# Autodesk Inventor assembly: N_core
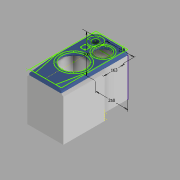
[picture p0: Inventor's stored thumbnail of the model, 180x180]
Saved by Autodesk Inventor 2022 (Build 260153000, 153)
## iProperties
Created: 2021-11-16
Part Number: N_core
Document SubType Name: Assembly
Designer: kalugin_a
Mass: 30078.3 g
Surface Area: 26443.9 cm^2
Volume: 21974.1 cm^3
Density: 1.36881 g/cm^3
Author: kalugin_a
## Documents named in this file (17)
- C:\Users\A\Documents\GitHub\Melas-DIII-base\Workspace\N_core.iam
- C:\Users\A\Documents\GitHub\Melas-DIII-base\Workspace\N_Front.ipt
- C:\Users\A\Documents\GitHub\Melas-DIII-base\Workspace\N_into_side.ipt
- C:\Users\A\Documents\GitHub\Melas-DIII-base\Workspace\N-Back_into.ipt
- C:\Users\A\Documents\GitHub\Melas-DIII-base\Workspace\N_Bottom.ipt
- C:\Users\A\Documents\GitHub\Melas-DIII-base\Workspace\MID.ipt
- C:\Users\A\Documents\GitHub\Melas-DIII-base\Workspace\N__side_sticker.ipt
- C:\Users\A\Documents\GitHub\Melas-DIII-base\Workspace\N__side_sticker_MIR.ipt
- C:\Users\A\Documents\GitHub\Melas-DIII-base\Workspace\WOOFER.ipt
- C:\Users\A\Documents\GitHub\Melas-DIII-base\Workspace\MIDRange.ipt
- C:\Users\A\Documents\GitHub\Melas-DIII-base\Workspace\Twitter.iam
- C:\Users\A\Documents\GitHub\Melas-DIII-base\Workspace\TopCover.ipt
- C:\Users\A\Documents\GitHub\Melas-DIII-base\Workspace\PowerSupply.ipt
- C:\Users\A\Documents\GitHub\Melas-DIII-base\Workspace\midwall-0.ipt
- C:\Users\A\Documents\GitHub\Melas-DIII-base\Workspace\FakeV.ipt
- C:\Users\A\Documents\GitHub\Melas-DIII-base\Workspace\ArmDesk.ipt
- C:\Users\A\Documents\GitHub\Melas-DIII-base\Workspace\motorDesk.ipt
## Components (18 placed, 17 different names)
1. N_Front:1 — Жесткий:18
2. N_into_side:1 — Жесткий:2, Жесткий:7, Совмещение:1
3. N_into_side:2 — Жесткий:1
4. N-Back_into:1 — Жесткий:14, Жесткий:15, Жесткий:16, Жесткий:17
5. N_Flane_H — Жесткий:15
6. MID:1
7. N__side_sticker:1 — Жесткий:17
8. N__side_sticker_MIR:1 — Жесткий:14
9. N_Bottom:3 — Жесткий:1, Жесткий:2, Жесткий:16, Жесткий:18
10. TopCover:1 — Жесткий:7
11. PowerSupply:1
12. midwall-0:1 — Жесткий:12
13. FakeV:1 — Жесткий:12
14. ArmDesk:1
15. motorDesk:1 — Совмещение:1
16. Twitter:1 [sub-assembly]
17. MIDRange:1
18. WOOFER:2
## Relationships (10: WeldJoint 9, Mate 1)
- Жесткий:1 [WeldJoint]: N_into_side:2 ↔ N_Bottom:3
- Жесткий:2 [WeldJoint]: N_into_side:1 ↔ N_Bottom:3
- Жесткий:7 [WeldJoint]: N_into_side:1 ↔ TopCover:1
- Жесткий:12 [WeldJoint]: midwall-0:1 ↔ FakeV:1
- Жесткий:14 [WeldJoint]: N-Back_into:1 ↔ N__side_sticker_MIR:1
- Жесткий:15 [WeldJoint]: N-Back_into:1 ↔ N_Flane_H
- Жесткий:16 [WeldJoint]: N-Back_into:1 ↔ N_Bottom:3
- Жесткий:17 [WeldJoint]: N-Back_into:1 ↔ N__side_sticker:1
- Жесткий:18 [WeldJoint]: N_Front:1 ↔ N_Bottom:3
- Совмещение:1 [Mate]: N_into_side:1 ↔ motorDesk:1
